# Autodesk Inventor assembly: X_Führung
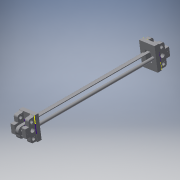
[picture p0: Inventor's stored thumbnail of the model, 180x180]
Saved by Autodesk Inventor 2019 (Build 230136000, 136)
## iProperties
Created: 2018-08-19
Part Number: X_Führung
Document SubType Name: Assembly
Designer: Julia
Author: Julia
## Documents named in this file (4)
- C:\Users\Julia\Documents\Inventor\3D_Drucker_v01\X_Führung.iam
- C:\Users\Julia\Documents\Inventor\3D_Drucker_v01\Y_Slider.iam
- C:\Users\Julia\Documents\Inventor\3D_Drucker_v01\X_Führungsstange.ipt
- C:\Users\Julia\Documents\Inventor\3D_Drucker_v01\X_Zahnriemen.ipt
## Components (5 placed, 3 different names)
1. Y_Slider:1 [sub-assembly] — Mate:1, Mate:2, Mate:7, Mate:8, Flush:1
2. Y_Slider:2 [sub-assembly] — Mate:3, Mate:4, Mate:5, Mate:6, Angle:1, Angle:2
3. X_Führungsstange:1 — Mate:2, Mate:4, Mate:5
4. X_Führungsstange:2 — Mate:1, Mate:3, Mate:6, Mate:7
5. X_Zahnriemen:1 — Angle:1, Angle:2, Mate:8, Flush:1
## Relationships (11: Mate 8, Angle 2, Flush 1)
- Mate:1: Y_Slider:1 ↔ X_Führungsstange:2
- Mate:2: Y_Slider:1 ↔ X_Führungsstange:1
- Mate:3: Y_Slider:2 ↔ X_Führungsstange:2
- Mate:4: Y_Slider:2 ↔ X_Führungsstange:1
- Mate:5: Y_Slider:2 ↔ X_Führungsstange:1
- Mate:6: Y_Slider:2 ↔ X_Führungsstange:2
- Mate:7: Y_Slider:1 ↔ X_Führungsstange:2
- Angle:1 (0 deg): Y_Slider:2 ↔ X_Zahnriemen:1
- Angle:2 (0 deg): Y_Slider:2 ↔ X_Zahnriemen:1
- Mate:8: Y_Slider:1 ↔ X_Zahnriemen:1
- Flush:1: Y_Slider:1 ↔ X_Zahnriemen:1
